# Autodesk Inventor assembly: E007_Boitier_v4_moduleElectronique
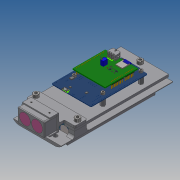
[picture p0: Inventor's stored thumbnail of the model, 180x180]
Saved by Autodesk Inventor 2021.3 (Build 253353000, 353)
## iProperties
Created: 2022-01-14
Part Number: E007_Boitier_v4_moduleElectronique
Document SubType Name: Assembly
Designer: gabri
Author: gabri
## Documents named in this file (14)
- D:\PGA\E007_Boitier_v4_moduleElectronique.iam
- D:\PGA\P040_BoitierCouvercleV4_module.ipt
- D:\PGA\Composants normalisés\18650 Battery.ipt
- D:\PGA\P042_BoitierCouvercleV4_moduleHaut.ipt
- D:\PGA\P043_entretoise15par3.ipt
- C:\Users\gabri\Documents\Inventor\Content Center Files\R2021\en-US\ISO 10642(2)\ISO 10642  - M3  x  8.ipt
- D:\PGA\P047_BoitierCouvercleV4_porteLidar.ipt
- D:\PGA\P041_Lidar.ipt
- C:\Users\gabri\Documents\Inventor\Content Center Files\R2021\en-US\ISO 4026\ISO 4026 - M3 x 2 - ISO.ipt
- C:\Users\gabri\Documents\Inventor\Content Center Files\R2021\en-US\BS EN ISO 4762\BS EN ISO 4762 - M5 x 12(1).ipt
- D:\PGA\Composants normalisés\ShieldLoRaSnow_shield.iam
- D:\PGA\Composants normalisés\B-L072Z-LRWAN1.iam
- C:\Users\gabri\Documents\Inventor\Content Center Files\R2021\en-US\BS EN ISO 4762\BS EN ISO 4762 - M3 x 8(1).ipt
- C:\Users\gabri\Documents\Inventor\Content Center Files\R2021\en-US\BS EN ISO 4762\BS EN ISO 4762 - M5 x 16(1).ipt
## Components (31 placed, 13 different names)
1. P040_BoitierCouvercleV4_module:1 — Mate:1, Mate:2, Mate:3, Mate:4, Mate:5, Mate:6, Mate:7, Mate:8, Mate:9, Mate:10, Mate:11, Mate:12, Mate:13, Mate:14, Mate:15, Mate:16, Mate:45, Mate:46
2. 18650 Battery:1 — Mate:6, Mate:11
3. 18650 Battery:2 — Mate:7, Mate:14
4. 18650 Battery:3 — Mate:4, Mate:12
5. 18650 Battery:4 — Mate:5
6. 18650 Battery:5 — Mate:9, Mate:10
7. 18650 Battery:6 — Mate:8, Mate:13
8. P042_BoitierCouvercleV4_moduleHaut:1 — Mate:15, Mate:16, Insert:1, Insert:2, Insert:3, Insert:4, Mate:18, Mate:22, Mate:23, Mate:24, Mate:26, Insert:7
9. P043_entretoise15par3:1 — Mate:17, Mate:18, Mate:44
10. DIN EN ISO 10642 M3  x  8:1 — Insert:3, Mate:19
11. DIN EN ISO 10642 M3  x  8:2 — Insert:1, Mate:20
12. DIN EN ISO 10642 M3  x  8:3 — Insert:4, Mate:21
13. DIN EN ISO 10642 M3  x  8:4 — Insert:2, Mate:17
14. P043_entretoise15par3:2 — Mate:19, Mate:22
15. P043_entretoise15par3:3 — Mate:20, Mate:24
16. P043_entretoise15par3:4 — Mate:21, Mate:23, Mate:39, Mate:40
17. P047_BoitierCouvercleV4_porteLidar:1 — Mate:26, Mate:29, Mate:30, Flush:1, Mate:31, Mate:32, Mate:33, Mate:34, Mate:36, Mate:37, Mate:38, Mate:45, Mate:46, Insert:14, Insert:15
18. P041_Lidar:1 — Mate:29, Mate:30, Flush:1, Mate:35
19. ISO 4026 M3 x 2:1 — Mate:33, Mate:37
20. ISO 4026 M3 x 2:2 — Mate:34, Mate:38
21. ISO 4026 M3 x 2:3 — Mate:31, Mate:36
22. ISO 4026 M3 x 2:4 — Mate:32, Mate:35
23. BS EN ISO 4762 - Metric M5 x 12:3 — Insert:7
24. ShieldLoRaSnow_shield:1 [sub-assembly] — Mate:41, Mate:42, Mate:43
25. B-L072Z-LRWAN1:1 [sub-assembly] — Mate:39, Mate:40, Mate:41, Mate:42, Mate:43, Mate:44, Insert:10, Insert:11, Insert:12, Insert:13
26. BS EN ISO 4762 - Metric M3 x 8:3 — Insert:10
27. BS EN ISO 4762 - Metric M3 x 8:4 — Insert:11
28. BS EN ISO 4762 - Metric M3 x 8:5 — Insert:13
29. BS EN ISO 4762 - Metric M3 x 8:6 — Insert:12
30. BS EN ISO 4762 - Metric M5 x 16:1 — Insert:15
31. BS EN ISO 4762 - Metric M5 x 16:2 — Insert:14
## Relationships (55: Mate 43, Insert 11, Flush 1)
- Mate:1: P040_BoitierCouvercleV4_module:1
- Mate:2: P040_BoitierCouvercleV4_module:1
- Mate:3: P040_BoitierCouvercleV4_module:1
- Mate:4: P040_BoitierCouvercleV4_module:1 ↔ 18650 Battery:3
- Mate:5: P040_BoitierCouvercleV4_module:1 ↔ 18650 Battery:4
- Mate:6: P040_BoitierCouvercleV4_module:1 ↔ 18650 Battery:1
- Mate:7: P040_BoitierCouvercleV4_module:1 ↔ 18650 Battery:2
- Mate:8: P040_BoitierCouvercleV4_module:1 ↔ 18650 Battery:6
- Mate:9: P040_BoitierCouvercleV4_module:1 ↔ 18650 Battery:5
- Mate:10 (3 mm): P040_BoitierCouvercleV4_module:1 ↔ 18650 Battery:5
- Mate:11 (3 mm): P040_BoitierCouvercleV4_module:1 ↔ 18650 Battery:1
- Mate:12 (3 mm): P040_BoitierCouvercleV4_module:1 ↔ 18650 Battery:3
- Mate:13 (3 mm): P040_BoitierCouvercleV4_module:1 ↔ 18650 Battery:6
- Mate:14 (3 mm): P040_BoitierCouvercleV4_module:1 ↔ 18650 Battery:2
- Mate:15: P040_BoitierCouvercleV4_module:1 ↔ P042_BoitierCouvercleV4_moduleHaut:1
- Mate:16: P040_BoitierCouvercleV4_module:1 ↔ P042_BoitierCouvercleV4_moduleHaut:1
- Insert:1: P042_BoitierCouvercleV4_moduleHaut:1 ↔ DIN EN ISO 10642 M3  x  8:2
- Insert:2: P042_BoitierCouvercleV4_moduleHaut:1 ↔ DIN EN ISO 10642 M3  x  8:4
- Insert:3: P042_BoitierCouvercleV4_moduleHaut:1 ↔ DIN EN ISO 10642 M3  x  8:1
- Insert:4: P042_BoitierCouvercleV4_moduleHaut:1 ↔ DIN EN ISO 10642 M3  x  8:3
- Mate:17: P043_entretoise15par3:1 ↔ DIN EN ISO 10642 M3  x  8:4
- Mate:18: P042_BoitierCouvercleV4_moduleHaut:1 ↔ P043_entretoise15par3:1
- Mate:19: DIN EN ISO 10642 M3  x  8:1 ↔ P043_entretoise15par3:2
- Mate:20: DIN EN ISO 10642 M3  x  8:2 ↔ P043_entretoise15par3:3
- Mate:21: DIN EN ISO 10642 M3  x  8:3 ↔ P043_entretoise15par3:4
- Mate:22: P042_BoitierCouvercleV4_moduleHaut:1 ↔ P043_entretoise15par3:2
- Mate:23: P042_BoitierCouvercleV4_moduleHaut:1 ↔ P043_entretoise15par3:4
- Mate:24: P042_BoitierCouvercleV4_moduleHaut:1 ↔ P043_entretoise15par3:3
- Mate:26: P042_BoitierCouvercleV4_moduleHaut:1 ↔ P047_BoitierCouvercleV4_porteLidar:1
- Mate:29: P047_BoitierCouvercleV4_porteLidar:1 ↔ P041_Lidar:1
- Mate:30: P047_BoitierCouvercleV4_porteLidar:1 ↔ P041_Lidar:1
- Flush:1 (-0.25 mm): P047_BoitierCouvercleV4_porteLidar:1 ↔ P041_Lidar:1
- Mate:31: P047_BoitierCouvercleV4_porteLidar:1 ↔ ISO 4026 M3 x 2:3
- Mate:32: P047_BoitierCouvercleV4_porteLidar:1 ↔ ISO 4026 M3 x 2:4
- Mate:33: P047_BoitierCouvercleV4_porteLidar:1 ↔ ISO 4026 M3 x 2:1
- Mate:34: P047_BoitierCouvercleV4_porteLidar:1 ↔ ISO 4026 M3 x 2:2
- Mate:35: P041_Lidar:1 ↔ ISO 4026 M3 x 2:4
- Mate:36: P047_BoitierCouvercleV4_porteLidar:1 ↔ ISO 4026 M3 x 2:3
- Mate:37: P047_BoitierCouvercleV4_porteLidar:1 ↔ ISO 4026 M3 x 2:1
- Mate:38: P047_BoitierCouvercleV4_porteLidar:1 ↔ ISO 4026 M3 x 2:2
- Insert:7: P042_BoitierCouvercleV4_moduleHaut:1 ↔ BS EN ISO 4762 - Metric M5 x 12:3
- Mate:39: P043_entretoise15par3:4 ↔ B-L072Z-LRWAN1:1
- Mate:40: P043_entretoise15par3:4 ↔ B-L072Z-LRWAN1:1
- Mate:41: ShieldLoRaSnow_shield:1 ↔ B-L072Z-LRWAN1:1
- Mate:42: ShieldLoRaSnow_shield:1 ↔ B-L072Z-LRWAN1:1
- Mate:43: ShieldLoRaSnow_shield:1 ↔ B-L072Z-LRWAN1:1
- Mate:44: P043_entretoise15par3:1 ↔ B-L072Z-LRWAN1:1
- Insert:10: B-L072Z-LRWAN1:1 ↔ BS EN ISO 4762 - Metric M3 x 8:3
- Insert:11: B-L072Z-LRWAN1:1 ↔ BS EN ISO 4762 - Metric M3 x 8:4
- Insert:12: B-L072Z-LRWAN1:1 ↔ BS EN ISO 4762 - Metric M3 x 8:6
- Insert:13: B-L072Z-LRWAN1:1 ↔ BS EN ISO 4762 - Metric M3 x 8:5
- Mate:45: P040_BoitierCouvercleV4_module:1 ↔ P047_BoitierCouvercleV4_porteLidar:1
- Mate:46: P040_BoitierCouvercleV4_module:1 ↔ P047_BoitierCouvercleV4_porteLidar:1
- Insert:14: P047_BoitierCouvercleV4_porteLidar:1 ↔ BS EN ISO 4762 - Metric M5 x 16:2
- Insert:15: P047_BoitierCouvercleV4_porteLidar:1 ↔ BS EN ISO 4762 - Metric M5 x 16:1
